# Autodesk Inventor assembly: motor unit
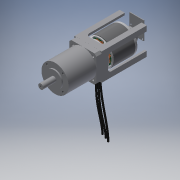
[picture p0: Inventor's stored thumbnail of the model, 180x180]
Saved by Autodesk Inventor 2018 (Build 220112000, 112)
## iProperties
Created: 2019-12-10
Part Number: motor unit
Document SubType Name: Assembly
Designer: Bunny320
Author: Bunny320
## Documents named in this file (7)
- C:\Users\Bunny320\Desktop\sechs\4-CAD\motor unit.iam
- C:\Users\Bunny320\Desktop\sechs\4-CAD\901-4250 house.ipt
- C:\Users\Bunny320\Desktop\sechs\4-CAD\911-42-reducer-long.ipt
- C:\Users\Bunny320\Desktop\sechs\4-CAD\standardParts\turnigy sk3 4250 350kv\BLDC Motor Turnigy Aerodrive SK3 350KV Outrunner.iam
- C:\Users\Bunny320\Desktop\sechs\4-CAD\902-4250 magnet hold.ipt
- C:\Users\Bunny320\Desktop\sechs\4-CAD\magnet-6x2.5.ipt
- C:\Users\Bunny320\Desktop\sechs\4-CAD\AS5047.ipt
## Components (6 placed, 6 different names)
1. 901-4250 house:1 — Flush:1, Flush:2, Flush:3, Mate:1, Mate:2, Mate:3, Mate:4, Flush:4
2. 911-42-reducer-long:1 — Mate:3, Mate:4, Flush:4
3. BLDC Motor Turnigy Aerodrive SK3 350KV Outrunner:1 [sub-assembly] — Mate:1, Mate:2, Mate:5, Mate:6
4. 902-4250 magnet hold:1 — Mate:5, Mate:6, Mate:7, Mate:8
5. magnet-6x2.5:1 — Mate:7, Mate:8, Mate:9
6. AS5047:1 — Mate:9
## Relationships (13: Mate 9, Flush 4)
- Flush:1: 901-4250 house:1
- Flush:2: 901-4250 house:1
- Flush:3: 901-4250 house:1
- Mate:1: 901-4250 house:1 ↔ BLDC Motor Turnigy Aerodrive SK3 350KV Outrunner:1
- Mate:2: 901-4250 house:1 ↔ BLDC Motor Turnigy Aerodrive SK3 350KV Outrunner:1
- Mate:3: 901-4250 house:1 ↔ 911-42-reducer-long:1
- Mate:4: 901-4250 house:1 ↔ 911-42-reducer-long:1
- Flush:4: 901-4250 house:1 ↔ 911-42-reducer-long:1
- Mate:5: BLDC Motor Turnigy Aerodrive SK3 350KV Outrunner:1 ↔ 902-4250 magnet hold:1
- Mate:6: BLDC Motor Turnigy Aerodrive SK3 350KV Outrunner:1 ↔ 902-4250 magnet hold:1
- Mate:7: 902-4250 magnet hold:1 ↔ magnet-6x2.5:1
- Mate:8: 902-4250 magnet hold:1 ↔ magnet-6x2.5:1
- Mate:9 (1.5 mm): magnet-6x2.5:1 ↔ AS5047:1
